# Autodesk Inventor assembly: LR_0311Full Pull Drawer1
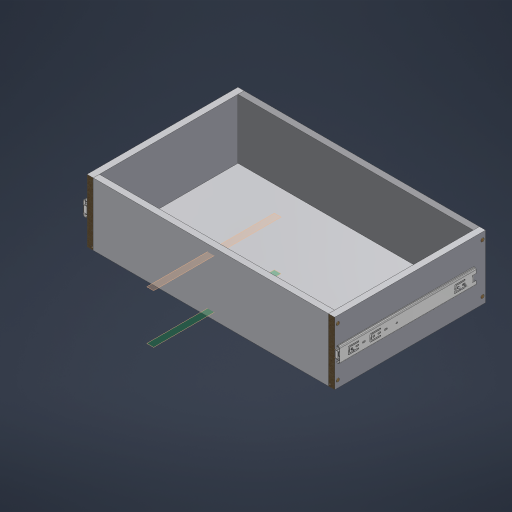
[picture p0: Inventor's stored thumbnail of the model, 512x512]
Saved by Autodesk Inventor 2024.3 (Build 283343000, 343)
## iProperties
Created: 2013-11-19
Part Number: LR_0311Full Pull Drawer1
Document SubType Name: Assembly
Designer: SauliusD
Description: Full Pull Drawer
Material Code: Item.FillWorkpiece.Material.Code
Author: SauliusD
## Documents named in this file (10)
- C:\W4INV 2024 Design\PROJECTS\Living Room\Commode\LR_03\iCopy\iCopy1\LR_0311Full Pull Drawer1.iam
- C:\W4INV 2024 Design\PROJECTS\Samples\Living Room\Commode\LR_03\iCopy\iCopy1\LR_0311DR Left1.ipt
- C:\W4INV 2024 Design\PROJECTS\Samples\Living Room\Commode\LR_03\iCopy\iCopy1\LR_0311DR Right1.ipt
- C:\W4INV 2024 Design\PROJECTS\Samples\Living Room\Commode\LR_03\iCopy\iCopy1\LR_0311DR Back1.ipt
- C:\W4INV 2024 Design\PROJECTS\Samples\Living Room\Commode\LR_03\iCopy\iCopy1\LR_0311DR Front1.ipt
- C:\W4INV 2024 Design\PROJECTS\Samples\Living Room\Commode\LR_03\iCopy\iCopy1\LR_0311DR Bottom1.ipt
- C:\W4INV 2024 Design\PROJECTS\Samples\Living Room\Commode\LR_03\iCopy\iCopy1\LR_0311Full Extension Ball bearing Slide1.iam
- C:\W4INV 2024 Design\_LIBRARY\Fixed joints\Confirmat\CONFIRMAT\Confirmat L50 & Cap D10 NB T18 PB T 18.ipt
- C:\W4INV 2024 Design\PROJECTS\Samples\Living Room\Commode\LR_03\iCopy\iCopy1\LR_0311Full Pull Drawer1.ipt
- C:\W4INV 2024 Design\LIBRARY\Fixed joints\Confirmat\CONFIRMAT.ipt
## Components (16 placed, 8 different names)
1. LR_0311Full Pull Drawer1:1 — Flush:16, Flush:17, Flush:18
2. LR_0311Full Extension Ball bearing Slide1:1 [sub-assembly] — Flush:2, Flush:3, Flush:4, Flush:5
3. LR_0311DR Left1:1 — Mate:1, Flush:1, Flush:8, Flush:10, Flush:12, Flush:14
4. LR_0311DR Right1:1 — Flush:9, Flush:11, Flush:13, Flush:15
5. LR_0311DR Back1:1 — Mate:7, Mate:9, Mate:15, Mate:17
6. LR_0311DR Front1:1 — Flush:6, Flush:7, Mate:3, Mate:5, Mate:11, Mate:13
7. LR_0311DR Bottom1:1
8. LR_0311Full Extension Ball bearing Slide1:2 [sub-assembly] — Mate:1, Flush:1, Flush:2
9. Confirmat L50 & Cap D10 NB T18 PB T 18:2 — Mate:2, Mate:3, Flush:8
10. Confirmat L50 & Cap D10 NB T18 PB T 18:3 — Mate:4, Mate:5, Flush:9
11. Confirmat L50 & Cap D10 NB T18 PB T 18:4 — Mate:6, Mate:7, Flush:10
12. Confirmat L50 & Cap D10 NB T18 PB T 18:5 — Mate:8, Mate:9, Flush:11
13. Confirmat L50 & Cap D10 NB T18 PB T 18:6 — Mate:10, Mate:11, Flush:12
14. Confirmat L50 & Cap D10 NB T18 PB T 18:7 — Mate:12, Mate:13, Flush:13
15. Confirmat L50 & Cap D10 NB T18 PB T 18:8 — Mate:14, Mate:15, Flush:14
16. Confirmat L50 & Cap D10 NB T18 PB T 18:9 — Mate:16, Mate:17, Flush:15
## Relationships (35: Flush 18, Mate 17)
- Mate:1: LR_0311DR Left1:1 ↔ LR_0311Full Extension Ball bearing Slide1:2
- Flush:1: LR_0311DR Left1:1 ↔ LR_0311Full Extension Ball bearing Slide1:2
- Flush:2: LR_0311Full Extension Ball bearing Slide1:1 ↔ LR_0311Full Extension Ball bearing Slide1:2
- Flush:3: LR_0311Full Extension Ball bearing Slide1:1
- Flush:4: LR_0311Full Extension Ball bearing Slide1:1
- Flush:5: LR_0311Full Extension Ball bearing Slide1:1
- Flush:6 (-20 mm): LR_0311DR Front1:1
- Flush:7 (-20 mm): LR_0311DR Front1:1
- Mate:2: Confirmat L50 & Cap D10 NB T18 PB T 18:2
- Mate:3 (-9 mm): LR_0311DR Front1:1 ↔ Confirmat L50 & Cap D10 NB T18 PB T 18:2
- Flush:8: LR_0311DR Left1:1 ↔ Confirmat L50 & Cap D10 NB T18 PB T 18:2
- Mate:4: Confirmat L50 & Cap D10 NB T18 PB T 18:3
- Mate:5 (-9 mm): LR_0311DR Front1:1 ↔ Confirmat L50 & Cap D10 NB T18 PB T 18:3
- Flush:9: LR_0311DR Right1:1 ↔ Confirmat L50 & Cap D10 NB T18 PB T 18:3
- Mate:6: Confirmat L50 & Cap D10 NB T18 PB T 18:4
- Mate:7 (-9 mm): LR_0311DR Back1:1 ↔ Confirmat L50 & Cap D10 NB T18 PB T 18:4
- Flush:10: LR_0311DR Left1:1 ↔ Confirmat L50 & Cap D10 NB T18 PB T 18:4
- Mate:8: Confirmat L50 & Cap D10 NB T18 PB T 18:5
- Mate:9 (-9 mm): LR_0311DR Back1:1 ↔ Confirmat L50 & Cap D10 NB T18 PB T 18:5
- Flush:11: LR_0311DR Right1:1 ↔ Confirmat L50 & Cap D10 NB T18 PB T 18:5
- Mate:10: Confirmat L50 & Cap D10 NB T18 PB T 18:6
- Mate:11 (-9 mm): LR_0311DR Front1:1 ↔ Confirmat L50 & Cap D10 NB T18 PB T 18:6
- Flush:12: LR_0311DR Left1:1 ↔ Confirmat L50 & Cap D10 NB T18 PB T 18:6
- Mate:12: Confirmat L50 & Cap D10 NB T18 PB T 18:7
- Mate:13 (-9 mm): LR_0311DR Front1:1 ↔ Confirmat L50 & Cap D10 NB T18 PB T 18:7
- Flush:13: LR_0311DR Right1:1 ↔ Confirmat L50 & Cap D10 NB T18 PB T 18:7
- Mate:14: Confirmat L50 & Cap D10 NB T18 PB T 18:8
- Mate:15 (-9 mm): LR_0311DR Back1:1 ↔ Confirmat L50 & Cap D10 NB T18 PB T 18:8
- Flush:14: LR_0311DR Left1:1 ↔ Confirmat L50 & Cap D10 NB T18 PB T 18:8
- Mate:16: Confirmat L50 & Cap D10 NB T18 PB T 18:9
- Mate:17 (-9 mm): LR_0311DR Back1:1 ↔ Confirmat L50 & Cap D10 NB T18 PB T 18:9
- Flush:15: LR_0311DR Right1:1 ↔ Confirmat L50 & Cap D10 NB T18 PB T 18:9
- Flush:16: LR_0311Full Pull Drawer1:1
- Flush:17: LR_0311Full Pull Drawer1:1
- Flush:18: LR_0311Full Pull Drawer1:1
## Named parameters: Inlet_Drawer = 0 mm
